# Autodesk Inventor assembly: Gen2Plate
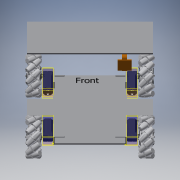
[picture p0: Inventor's stored thumbnail of the model, 180x180]
Saved by Autodesk Inventor 2017 (Build 210142000, 142)
## iProperties
Created: 2017-12-06
Part Number: Gen2Plate
Document SubType Name: Assembly
Designer: User
Author: User
## Documents named in this file (7)
- C:\Robotics\CAD\2017-18_CAD\Prototypes\Gen2Plate.iam
- C:\Robotics\CAD\2017-18_CAD\Prototypes\Gen2PlatePart.ipt
- C:\Robotics\CAD\2017-18_CAD\Prototypes\HexMotorDirectDrive.iam
- C:\Robotics\CAD\2017-18_CAD\Prototypes\MecanumWheelFullForVexmotor.iam
- C:\Robotics\CAD\COTSParts\Rev\REV-41-1300.ipt
- C:\Robotics\CAD\2017-18_CAD\Phone_Cas.ipt
- C:\Robotics\CAD\2017-18_CAD\Prototypes\PossibleTopPlate.ipt
## Components (10 placed, 6 different names)
1. Gen2PlatePart:1 — Mate:1, Mate:2, Mate:8, Mate:9, Mate:10, Flush:11, Mate:11, Mate:12, Mate:13, Mate:14, Mate:17, Mate:18, Flush:14, Flush:15, Flush:16, Mate:19, Flush:18, Flush:19
2. HexMotorDirectDrive:1 [sub-assembly] — Mate:1, Flush:10, Flush:12, Mate:17, Mate:18
3. MecanumWheelFullForVexmotor:1 [sub-assembly] — Mate:6, Mate:7, Flush:12
4. MecanumWheelFullForVexmotor:2 [sub-assembly] — Mate:3, Mate:4, Mate:5, Flush:10, Flush:13
5. MecanumWheelFullForVexmotor:3 [sub-assembly] — Mate:15, Mate:16, Flush:13
6. REV-41-1300:2 — Mate:11, Mate:12, Mate:13, Mate:15, Mate:16
7. REV-41-1300:3 — Mate:6, Mate:7, Mate:8, Mate:14
8. REV-41-1300:4 — Mate:2, Mate:3, Mate:4, Mate:5, Mate:9, Mate:10, Flush:11
9. Phone_Cas:4 — Flush:14, Flush:15, Flush:16
10. PossibleTopPlate:1 — Mate:19, Flush:18, Flush:19
## Relationships (28: Mate 19, Flush 9)
- Mate:1: Gen2PlatePart:1 ↔ HexMotorDirectDrive:1
- Mate:2: Gen2PlatePart:1 ↔ REV-41-1300:4
- Mate:3: MecanumWheelFullForVexmotor:2 ↔ REV-41-1300:4
- Mate:4: MecanumWheelFullForVexmotor:2 ↔ REV-41-1300:4
- Mate:5 (7.0104 mm): MecanumWheelFullForVexmotor:2 ↔ REV-41-1300:4
- Mate:6: MecanumWheelFullForVexmotor:1 ↔ REV-41-1300:3
- Mate:7: MecanumWheelFullForVexmotor:1 ↔ REV-41-1300:3
- Flush:10: HexMotorDirectDrive:1 ↔ MecanumWheelFullForVexmotor:2
- Mate:8: Gen2PlatePart:1 ↔ REV-41-1300:3
- Mate:9: Gen2PlatePart:1 ↔ REV-41-1300:4
- Mate:10: Gen2PlatePart:1 ↔ REV-41-1300:4
- Flush:11: Gen2PlatePart:1 ↔ REV-41-1300:4
- Mate:11: Gen2PlatePart:1 ↔ REV-41-1300:2
- Mate:12: Gen2PlatePart:1 ↔ REV-41-1300:2
- Mate:13: Gen2PlatePart:1 ↔ REV-41-1300:2
- Flush:12: HexMotorDirectDrive:1 ↔ MecanumWheelFullForVexmotor:1
- Mate:14: Gen2PlatePart:1 ↔ REV-41-1300:3
- Mate:15: MecanumWheelFullForVexmotor:3 ↔ REV-41-1300:2
- Mate:16: MecanumWheelFullForVexmotor:3 ↔ REV-41-1300:2
- Flush:13: MecanumWheelFullForVexmotor:2 ↔ MecanumWheelFullForVexmotor:3
- Mate:17: Gen2PlatePart:1 ↔ HexMotorDirectDrive:1
- Mate:18: Gen2PlatePart:1 ↔ HexMotorDirectDrive:1
- Flush:14 (-210.7692 mm): Gen2PlatePart:1 ↔ Phone_Cas:4
- Flush:15 (-12.7 mm): Gen2PlatePart:1 ↔ Phone_Cas:4
- Flush:16: Gen2PlatePart:1 ↔ Phone_Cas:4
- Mate:19 (254 mm): Gen2PlatePart:1 ↔ PossibleTopPlate:1
- Flush:18: Gen2PlatePart:1 ↔ PossibleTopPlate:1
- Flush:19: Gen2PlatePart:1 ↔ PossibleTopPlate:1
